# Autodesk Inventor assembly: ropeDriver
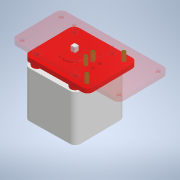
[picture p0: Inventor's stored thumbnail of the model, 180x180]
Saved by Autodesk Inventor 2020 (Build 240168000, 168)
## iProperties
Created: 2020-02-03
Part Number: ropeDriver
Document SubType Name: Assembly
Designer: Felix
Author: Felix
## Documents named in this file (6)
- C:\Users\Felix\Documents\Programmieren\ropeBot\testBotV1\ropeDriver.iam
- C:\Users\Felix\Documents\Programmieren\ropeBot\testBotV1\stepper.ipt
- C:\Users\Felix\Documents\Programmieren\ropeBot\testBotV1\housing.ipt
- C:\Users\Felix\Documents\Programmieren\ropeBot\testBotV1\brassPin.ipt
- C:\Users\Felix\Documents\Programmieren\ropeBot\testBotV1\pulley.ipt
- C:\Users\Felix\Documents\Programmieren\ropeBot\testBotV1\housingBack.ipt
## Components (8 placed, 5 different names)
1. stepper:1 — Mate:2, Mate:9
2. housing:1 — Mate:1, Flush:2, Flush:3, Mate:5, Flush:4, Flush:5, Flush:6, Mate:6, Mate:7, Mate:8, Mate:9, Mate:10, Mate:11
3. brassPin:1 — Mate:1, Flush:2
4. pulley:1 — Flush:3, Mate:2
5. brassPin:2 — Flush:6, Mate:10
6. brassPin:3 — Flush:5, Mate:11
7. brassPin:4 — Mate:5, Flush:4
8. housingBack:1 — Mate:6, Mate:7, Mate:8
## Relationships (14: Mate 9, Flush 5)
- Mate:1: housing:1 ↔ brassPin:1
- Flush:2: housing:1 ↔ brassPin:1
- Flush:3 (0.5 mm): housing:1 ↔ pulley:1
- Mate:2: stepper:1 ↔ pulley:1
- Mate:5: housing:1 ↔ brassPin:4
- Flush:4: housing:1 ↔ brassPin:4
- Flush:5: housing:1 ↔ brassPin:3
- Flush:6: housing:1 ↔ brassPin:2
- Mate:6: housing:1 ↔ housingBack:1
- Mate:7: housing:1 ↔ housingBack:1
- Mate:8: housing:1 ↔ housingBack:1
- Mate:9: stepper:1 ↔ housing:1
- Mate:10: housing:1 ↔ brassPin:2
- Mate:11: housing:1 ↔ brassPin:3
